# Autodesk Inventor assembly: Most_example
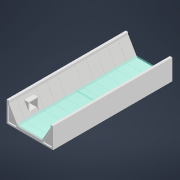
[picture p0: Inventor's stored thumbnail of the model, 180x180]
Saved by Autodesk Inventor 2022 (Build 260153000, 153)
## iProperties
Created: 2022-02-21
Part Number: Most_example
Document SubType Name: Assembly
Designer: Lukas
Author: Lukas
## Documents named in this file (4)
- C:\Users\Lukas\Desktop\ard\3D\Walle\Most_example.iam
- C:\Users\Lukas\Desktop\ard\3D\Walle\McCrea_Kanal_Walle.ipt
- C:\Users\Lukas\Desktop\ard\3D\Walle\McCrea_Kanal_diera_Walle.ipt
- C:\Users\Lukas\Desktop\ard\3D\Walle\watah.ipt
## Components (4 placed, 3 different names)
1. McCrea_Kanal_Walle:1 — Mate:1, Mate:2, Mate:6
2. McCrea_Kanal_diera_Walle:1 — Mate:1, Mate:2, Mate:3, Mate:4, Mate:5
3. watah:1 — Mate:3, Mate:4
4. watah:2 — Mate:5, Mate:6
## Relationships (6: Mate 6)
- Mate:1: McCrea_Kanal_Walle:1 ↔ McCrea_Kanal_diera_Walle:1
- Mate:2: McCrea_Kanal_Walle:1 ↔ McCrea_Kanal_diera_Walle:1
- Mate:3: McCrea_Kanal_diera_Walle:1 ↔ watah:1
- Mate:4: McCrea_Kanal_diera_Walle:1 ↔ watah:1
- Mate:5: McCrea_Kanal_diera_Walle:1 ↔ watah:2
- Mate:6: McCrea_Kanal_Walle:1 ↔ watah:2
